# Autodesk Inventor assembly: ROV
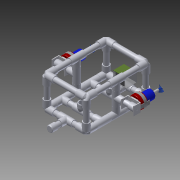
[picture p0: Inventor's stored thumbnail of the model, 180x180]
Saved by Autodesk Inventor 2013 (Build 170138000, 138)
## iProperties
Created: 2014-07-04
Part Number: ROV
Document SubType Name: Assembly
Designer: Kyle
Author: Kyle
## Documents named in this file (17)
- B:\Libraries\Documents\Autodesk\Output\Inventor 2013\ROV\ROV Gen 3.iam
- B:\Libraries\Documents\Autodesk\Output\Inventor 2013\ROV\0.5 3 Way.ipt
- B:\Libraries\Documents\Autodesk\Output\Inventor 2013\ROV\0.5 Tee.ipt
- B:\Libraries\Documents\Autodesk\Output\Inventor 2013\ROV\0.75 Pipe.ipt
- B:\Libraries\Documents\Autodesk\Output\Inventor 2013\ROV\Flush Connect Pipe.ipt
- B:\Libraries\Documents\Autodesk\Output\Inventor 2013\ROV\Cap.ipt
- B:\Libraries\Documents\Autodesk\Output\Inventor 2013\ROV\Cap Pipe.ipt
- B:\Libraries\Documents\Autodesk\Output\Inventor 2013\ROV\0.5 to 0.75 Tee.ipt
- B:\Libraries\Documents\Autodesk\Output\Inventor 2013\ROV\2 Pipe.ipt
- B:\Libraries\Documents\Autodesk\Output\Inventor 2013\ROV\2.75 Pipe.ipt
- B:\Libraries\Documents\Autodesk\Output\Inventor 2013\ROV\4 Pipe.ipt
- B:\Libraries\Documents\Autodesk\Output\Inventor 2013\ROV\2.4 Pipe.ipt
- B:\Libraries\Documents\Autodesk\Output\Inventor 2013\ROV\3 Pipe.ipt
- B:\Libraries\Documents\Autodesk\Output\Inventor 2013\ROV\Long Cap.ipt
- B:\Libraries\Documents\Autodesk\Output\Inventor 2013\ROV\Motor Assembly\Motor Bracket.iam
- B:\Libraries\Documents\Autodesk\Output\Inventor 2013\ROV\Long Cap .125 Hole.ipt
- B:\Libraries\Documents\Autodesk\Output\Inventor 2013\ROV\Box\Box.iam
## Components (63 placed, 16 different names)
1. 0.5 3 Way:1 — Mate:1, Mate:2, Angle:1, Flush:1, Mate:21, Mate:22, Mate:24, Angle:3, Angle:7, Mate:73, Mate:77
2. 0.5 3 Way:2 — Mate:7, Mate:8, Flush:1, Mate:13, Mate:14, Mate:20, Angle:2, Angle:4, Angle:8, Mate:72, Mate:76, Angle:19, Angle:22
3. 0.5 3 Way:3 — Mate:50, Mate:55, Angle:10, Mate:66, Mate:68, Mate:75, Mate:78, Angle:18
4. 0.5 3 Way:4 — Mate:51, Mate:54, Angle:9, Mate:67, Mate:69, Mate:74, Mate:79
5. 0.5 Tee:1 — Mate:3, Mate:4, Angle:1, Mate:5, Mate:6, Mate:15, Mate:16, Mate:18, Tangent:1, Flush:8
6. 0.5 Tee:2 — Mate:23, Mate:24, Angle:3, Mate:26, Mate:27, Mate:34, Mate:38
7. 0.5 Tee:3 — Mate:19, Mate:20, Angle:2, Mate:25, Mate:28, Mate:32, Mate:36
8. 0.75 Pipe:1 — Mate:1, Mate:2, Mate:3, Mate:4
9. 0.75 Pipe:2 — Mate:5, Mate:6, Mate:7, Mate:8
10. Flush Connect Pipe:2 — Mate:13, Mate:14, Mate:19
11. Flush Connect Pipe:3 — Mate:21, Mate:22, Mate:23
12. Cap Pipe:1 — Mate:15, Mate:16, Mate:17
13. Cap:1 — Mate:17, Mate:18
14. 0.75 Pipe:3 — Mate:26, Mate:27, Mate:30, Mate:31
15. 0.75 Pipe:4 — Mate:25, Mate:28, Mate:29
16. 0.5 to 0.75 Tee:1 — Mate:29, Mate:30, Mate:31, Angle:4, Angle:5, Angle:6, Angle:12
17. 0.5 Tee:4 — Mate:33, Mate:37, Angle:5, Mate:40, Mate:42, Angle:9, Mate:80, Mate:82
18. 0.5 Tee:5 — Mate:35, Mate:39, Angle:6, Mate:41, Mate:43, Angle:10, Mate:81, Mate:83
19. Flush Connect Pipe:4 — Mate:32, Mate:33, Mate:36, Mate:37
20. Flush Connect Pipe:5 — Mate:34, Mate:35, Mate:38, Mate:39
21. Flush Connect Pipe:6 — Mate:41, Mate:43, Mate:45, Mate:47
22. Flush Connect Pipe:7 — Mate:40, Mate:42, Mate:44, Mate:46
23. 0.5 Tee:6 — Mate:44, Mate:46, Angle:8, Mate:48, Mate:52, Mate:54, Angle:11
24. 0.5 Tee:7 — Mate:45, Mate:47, Angle:7, Mate:49, Mate:53, Mate:55, Mate:60, Angle:13
25. Flush Connect Pipe:8 — Mate:49, Mate:50, Mate:53
26. Flush Connect Pipe:9 — Mate:48, Mate:51, Mate:52
27. 0.5 to 0.75 Tee:2 — Mate:56, Mate:57, Mate:58, Angle:12, Mate:61, Angle:14, Angle:15
28. 0.75 Pipe:5 — Mate:56, Mate:58, Mate:60
29. 0.75 Pipe:6 — Mate:57, Angle:11, Mate:61
30. 0.75 Pipe:7 — Mate:66, Mate:68, Mate:70
31. 0.75 Pipe:8 — Mate:67, Mate:69, Mate:71
32. 0.5 Tee:8 — Mate:70, Mate:71, Angle:13, Mate:127, Mate:128
33. 2 Pipe:1 — Mate:72, Mate:76
34. 2 Pipe:2 — Mate:73, Mate:77
35. 2 Pipe:3 — Mate:75, Mate:78
36. 2 Pipe:4 — Mate:74, Mate:79
37. Flush Connect Pipe:10 — Mate:80, Mate:82, Mate:84, Mate:86
38. Flush Connect Pipe:11 — Mate:81, Mate:83, Mate:85, Mate:87
39. 0.5 Tee:9 — Mate:84, Mate:86, Angle:14, Mate:88, Mate:90, Mate:129, Mate:131
40. 0.5 Tee:10 — Mate:85, Mate:87, Angle:15, Mate:89, Mate:91, Mate:118, Mate:130, Mate:132
41. Flush Connect Pipe:12 — Mate:88, Mate:90, Mate:117
42. Flush Connect Pipe:13 — Mate:89, Mate:91
43. 0.5 3 Way:5 — Mate:112, Mate:113, Mate:114, Mate:115, Angle:18
44. 0.5 3 Way:6 — Mate:92, Mate:95, Mate:96, Mate:97, Flush:2, Angle:17
45. 0.5 3 Way:7 — Mate:98, Mate:99, Mate:100, Flush:2, Mate:101, Angle:16, Flush:3
46. 0.5 3 Way:8 — Mate:110, Mate:111, Flush:3, Mate:114, Mate:116
47. 2.75 Pipe:1 — Mate:92, Mate:95, Mate:103, Mate:105
48. 2.75 Pipe:2 — Mate:106, Mate:109, Mate:110, Mate:111
49. 2.75 Pipe:3 — Mate:107, Mate:108, Mate:112, Mate:113
50. 2.75 Pipe:4 — Mate:100, Mate:101, Mate:102, Mate:104
51. 4 Pipe:1 — Mate:96, Mate:97, Mate:98, Mate:99
52. 4 Pipe:2 — Mate:115, Mate:116
53. 0.5 Tee:11 — Mate:102, Angle:16, Mate:104, Mate:106, Mate:109, Mate:117
54. 0.5 Tee:12 — Mate:103, Angle:17, Mate:105, Mate:107, Mate:108, Mate:118
55. 2.4 Pipe:1 — Mate:127, Mate:128, Mate:133, Mate:134
56. 3 Pipe:1 — Mate:129, Mate:131, Mate:139, Mate:140, Mate:141
57. 3 Pipe:2 — Mate:130, Mate:132, Mate:142, Mate:143, Mate:145
58. Long Cap:1 — Mate:133, Mate:134
59. Motor Bracket:1 [sub-assembly] — Mate:139, Mate:144, Angle:19, Angle:20
60. Motor Bracket:2 [sub-assembly] — Mate:145, Mate:146, Angle:20, Angle:21, Mate:147
61. Long Cap .125 Hole:1 — Mate:140, Mate:141, Mate:144
62. Long Cap .125 Hole:2 — Mate:142, Mate:143, Mate:146
63. Box:1 [sub-assembly] — Tangent:1, Angle:21, Angle:22, Mate:147, Flush:8
## Relationships (151: Mate 124, Angle 22, Flush 4, Tangent 1)
- Mate:1: 0.5 3 Way:1 ↔ 0.75 Pipe:1
- Mate:2: 0.5 3 Way:1 ↔ 0.75 Pipe:1
- Mate:3: 0.5 Tee:1 ↔ 0.75 Pipe:1
- Mate:4: 0.5 Tee:1 ↔ 0.75 Pipe:1
- Angle:1 (0 deg): 0.5 3 Way:1 ↔ 0.5 Tee:1
- Mate:5: 0.5 Tee:1 ↔ 0.75 Pipe:2
- Mate:6: 0.5 Tee:1 ↔ 0.75 Pipe:2
- Mate:7: 0.5 3 Way:2 ↔ 0.75 Pipe:2
- Mate:8: 0.5 3 Way:2 ↔ 0.75 Pipe:2
- Flush:1: 0.5 3 Way:1 ↔ 0.5 3 Way:2
- Mate:13: 0.5 3 Way:2 ↔ Flush Connect Pipe:2
- Mate:14: 0.5 3 Way:2 ↔ Flush Connect Pipe:2
- Mate:15: 0.5 Tee:1 ↔ Cap Pipe:1
- Mate:16: 0.5 Tee:1 ↔ Cap Pipe:1
- Mate:17: Cap Pipe:1 ↔ Cap:1
- Mate:18: 0.5 Tee:1 ↔ Cap:1
- Mate:19: 0.5 Tee:3 ↔ Flush Connect Pipe:2
- Mate:20: 0.5 3 Way:2 ↔ 0.5 Tee:3
- Angle:2 (0 deg): 0.5 3 Way:2 ↔ 0.5 Tee:3
- Mate:21: 0.5 3 Way:1 ↔ Flush Connect Pipe:3
- Mate:22: 0.5 3 Way:1 ↔ Flush Connect Pipe:3
- Mate:23: 0.5 Tee:2 ↔ Flush Connect Pipe:3
- Mate:24: 0.5 3 Way:1 ↔ 0.5 Tee:2
- Angle:3 (0 deg): 0.5 3 Way:1 ↔ 0.5 Tee:2
- Mate:25: 0.5 Tee:3 ↔ 0.75 Pipe:4
- Mate:26: 0.5 Tee:2 ↔ 0.75 Pipe:3
- Mate:27: 0.5 Tee:2 ↔ 0.75 Pipe:3
- Mate:28: 0.5 Tee:3 ↔ 0.75 Pipe:4
- Mate:29: 0.75 Pipe:4 ↔ 0.5 to 0.75 Tee:1
- Mate:30: 0.75 Pipe:3 ↔ 0.5 to 0.75 Tee:1
- Mate:31: 0.75 Pipe:3 ↔ 0.5 to 0.75 Tee:1
- Angle:4 (0 deg): 0.5 3 Way:2 ↔ 0.5 to 0.75 Tee:1
- Mate:32: 0.5 Tee:3 ↔ Flush Connect Pipe:4
- Mate:33: 0.5 Tee:4 ↔ Flush Connect Pipe:4
- Mate:34: 0.5 Tee:2 ↔ Flush Connect Pipe:5
- Mate:35: 0.5 Tee:5 ↔ Flush Connect Pipe:5
- Mate:36: 0.5 Tee:3 ↔ Flush Connect Pipe:4
- Mate:37: 0.5 Tee:4 ↔ Flush Connect Pipe:4
- Mate:38: 0.5 Tee:2 ↔ Flush Connect Pipe:5
- Mate:39: 0.5 Tee:5 ↔ Flush Connect Pipe:5
- Angle:5 (0 deg): 0.5 to 0.75 Tee:1 ↔ 0.5 Tee:4
- Angle:6 (0 deg): 0.5 to 0.75 Tee:1 ↔ 0.5 Tee:5
- Mate:40: 0.5 Tee:4 ↔ Flush Connect Pipe:7
- Mate:41: 0.5 Tee:5 ↔ Flush Connect Pipe:6
- Mate:42: 0.5 Tee:4 ↔ Flush Connect Pipe:7
- Mate:43: 0.5 Tee:5 ↔ Flush Connect Pipe:6
- Mate:44: Flush Connect Pipe:7 ↔ 0.5 Tee:6
- Mate:45: Flush Connect Pipe:6 ↔ 0.5 Tee:7
- Mate:46: Flush Connect Pipe:7 ↔ 0.5 Tee:6
- Mate:47: Flush Connect Pipe:6 ↔ 0.5 Tee:7
- Angle:7 (0 deg): 0.5 3 Way:1 ↔ 0.5 Tee:7
- Angle:8 (0 deg): 0.5 3 Way:2 ↔ 0.5 Tee:6
- Mate:48: 0.5 Tee:6 ↔ Flush Connect Pipe:9
- Mate:49: 0.5 Tee:7 ↔ Flush Connect Pipe:8
- Mate:50: 0.5 3 Way:3 ↔ Flush Connect Pipe:8
- Mate:51: 0.5 3 Way:4 ↔ Flush Connect Pipe:9
- Mate:52: 0.5 Tee:6 ↔ Flush Connect Pipe:9
- Mate:53: 0.5 Tee:7 ↔ Flush Connect Pipe:8
- Mate:54: 0.5 3 Way:4 ↔ 0.5 Tee:6
- Mate:55: 0.5 3 Way:3 ↔ 0.5 Tee:7
- Angle:9 (0 deg): 0.5 3 Way:4 ↔ 0.5 Tee:4
- Angle:10 (0 deg): 0.5 3 Way:3 ↔ 0.5 Tee:5
- Mate:56: 0.5 to 0.75 Tee:2 ↔ 0.75 Pipe:5
- Mate:57: 0.5 to 0.75 Tee:2 ↔ 0.75 Pipe:6
- Mate:58: 0.5 to 0.75 Tee:2 ↔ 0.75 Pipe:5
- Mate:60: 0.5 Tee:7 ↔ 0.75 Pipe:5
- Angle:11 (0 deg): 0.5 Tee:6 ↔ 0.75 Pipe:6
- Angle:12 (0 deg): 0.5 to 0.75 Tee:1 ↔ 0.5 to 0.75 Tee:2
- Mate:61: 0.5 to 0.75 Tee:2 ↔ 0.75 Pipe:6
- Mate:66: 0.5 3 Way:3 ↔ 0.75 Pipe:7
- Mate:67: 0.5 3 Way:4 ↔ 0.75 Pipe:8
- Mate:68: 0.5 3 Way:3 ↔ 0.75 Pipe:7
- Mate:69: 0.5 3 Way:4 ↔ 0.75 Pipe:8
- Mate:70: 0.75 Pipe:7 ↔ 0.5 Tee:8
- Mate:71: 0.75 Pipe:8 ↔ 0.5 Tee:8
- Angle:13 (180 deg): 0.5 Tee:7 ↔ 0.5 Tee:8
- Mate:72: 0.5 3 Way:2 ↔ 2 Pipe:1
- Mate:73: 0.5 3 Way:1 ↔ 2 Pipe:2
- Mate:74: 0.5 3 Way:4 ↔ 2 Pipe:4
- Mate:75: 0.5 3 Way:3 ↔ 2 Pipe:3
- Mate:76: 0.5 3 Way:2 ↔ 2 Pipe:1
- Mate:77: 0.5 3 Way:1 ↔ 2 Pipe:2
- Mate:78: 0.5 3 Way:3 ↔ 2 Pipe:3
- Mate:79: 0.5 3 Way:4 ↔ 2 Pipe:4
- Mate:80: 0.5 Tee:4 ↔ Flush Connect Pipe:10
- Mate:81: 0.5 Tee:5 ↔ Flush Connect Pipe:11
- Mate:82: 0.5 Tee:4 ↔ Flush Connect Pipe:10
- Mate:83: 0.5 Tee:5 ↔ Flush Connect Pipe:11
- Mate:84: Flush Connect Pipe:10 ↔ 0.5 Tee:9
- Mate:85: Flush Connect Pipe:11 ↔ 0.5 Tee:10
- Mate:86: Flush Connect Pipe:10 ↔ 0.5 Tee:9
- Mate:87: Flush Connect Pipe:11 ↔ 0.5 Tee:10
- Angle:14 (0 deg): 0.5 to 0.75 Tee:2 ↔ 0.5 Tee:9
- Angle:15 (0 deg): 0.5 to 0.75 Tee:2 ↔ 0.5 Tee:10
- Mate:88: 0.5 Tee:9 ↔ Flush Connect Pipe:12
- Mate:89: 0.5 Tee:10 ↔ Flush Connect Pipe:13
- Mate:90: 0.5 Tee:9 ↔ Flush Connect Pipe:12
- Mate:91: 0.5 Tee:10 ↔ Flush Connect Pipe:13
- Mate:92: 0.5 3 Way:6 ↔ 2.75 Pipe:1
- Mate:95: 0.5 3 Way:6 ↔ 2.75 Pipe:1
- Mate:96: 0.5 3 Way:6 ↔ 4 Pipe:1
- Mate:97: 0.5 3 Way:6 ↔ 4 Pipe:1
- Mate:98: 0.5 3 Way:7 ↔ 4 Pipe:1
- Mate:99: 0.5 3 Way:7 ↔ 4 Pipe:1
- Mate:100: 0.5 3 Way:7 ↔ 2.75 Pipe:4
- Flush:2: 0.5 3 Way:6 ↔ 0.5 3 Way:7
- Mate:101: 0.5 3 Way:7 ↔ 2.75 Pipe:4
- Mate:102: 2.75 Pipe:4 ↔ 0.5 Tee:11
- Mate:103: 2.75 Pipe:1 ↔ 0.5 Tee:12
- Angle:16 (0 deg): 0.5 3 Way:7 ↔ 0.5 Tee:11
- Angle:17 (0 deg): 0.5 3 Way:6 ↔ 0.5 Tee:12
- Mate:104: 2.75 Pipe:4 ↔ 0.5 Tee:11
- Mate:105: 2.75 Pipe:1 ↔ 0.5 Tee:12
- Mate:106: 2.75 Pipe:2 ↔ 0.5 Tee:11
- Mate:107: 2.75 Pipe:3 ↔ 0.5 Tee:12
- Mate:108: 2.75 Pipe:3 ↔ 0.5 Tee:12
- Mate:109: 2.75 Pipe:2 ↔ 0.5 Tee:11
- Mate:110: 0.5 3 Way:8 ↔ 2.75 Pipe:2
- Mate:111: 0.5 3 Way:8 ↔ 2.75 Pipe:2
- Flush:3: 0.5 3 Way:7 ↔ 0.5 3 Way:8
- Mate:112: 0.5 3 Way:5 ↔ 2.75 Pipe:3
- Mate:113: 0.5 3 Way:5 ↔ 2.75 Pipe:3
- Mate:114: 0.5 3 Way:5 ↔ 0.5 3 Way:8
- Mate:115: 0.5 3 Way:5 ↔ 4 Pipe:2
- Mate:116: 0.5 3 Way:8 ↔ 4 Pipe:2
- Mate:117: Flush Connect Pipe:12 ↔ 0.5 Tee:11
- Angle:18 (0 deg): 0.5 3 Way:3 ↔ 0.5 3 Way:5
- Mate:118: 0.5 Tee:10 ↔ 0.5 Tee:12
- Mate:127: 0.5 Tee:8 ↔ 2.4 Pipe:1
- Mate:128: 0.5 Tee:8 ↔ 2.4 Pipe:1
- Mate:129: 0.5 Tee:9 ↔ 3 Pipe:1
- Mate:130: 0.5 Tee:10 ↔ 3 Pipe:2
- Mate:131: 0.5 Tee:9 ↔ 3 Pipe:1
- Mate:132: 0.5 Tee:10 ↔ 3 Pipe:2
- Mate:133: 2.4 Pipe:1 ↔ Long Cap:1
- Mate:134: 2.4 Pipe:1 ↔ Long Cap:1
- Mate:139: 3 Pipe:1 ↔ Motor Bracket:1
- Mate:140: 3 Pipe:1 ↔ Long Cap .125 Hole:1
- Mate:141: 3 Pipe:1 ↔ Long Cap .125 Hole:1
- Mate:142: 3 Pipe:2 ↔ Long Cap .125 Hole:2
- Mate:143: 3 Pipe:2 ↔ Long Cap .125 Hole:2
- Mate:144: Motor Bracket:1 ↔ Long Cap .125 Hole:1
- Angle:19 (0 deg): 0.5 3 Way:2 ↔ Motor Bracket:1
- Mate:145: 3 Pipe:2 ↔ Motor Bracket:2
- Mate:146: Motor Bracket:2 ↔ Long Cap .125 Hole:2
- Angle:20 (0 deg): Motor Bracket:1 ↔ Motor Bracket:2
- Tangent:1: 0.5 Tee:1 ↔ Box:1
- Angle:21 (0 deg): Motor Bracket:2 ↔ Box:1
- Angle:22 (0 deg): 0.5 3 Way:2 ↔ Box:1
- Mate:147 (12.7 mm): Motor Bracket:2 ↔ Box:1
- Flush:8 (-2.54 mm): 0.5 Tee:1 ↔ Box:1
